# Autodesk Inventor assembly: Pelvis
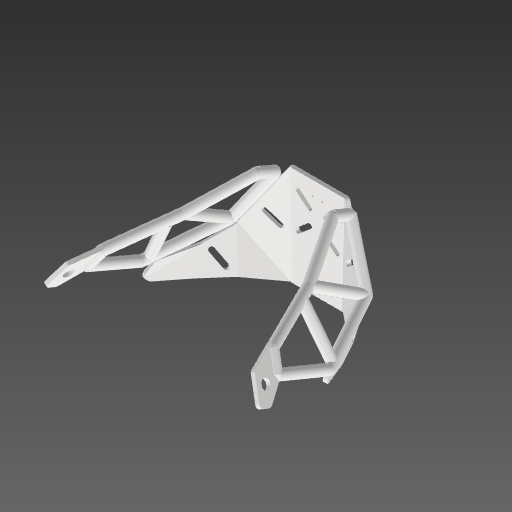
[picture p0: Inventor's stored thumbnail of the model, 512x512]
Saved by Autodesk Inventor 2020 (Build 240168000, 168)
## iProperties
Created: 2020-05-05
Part Number: Pelvis
Document SubType Name: Assembly
Designer: valer
Author: valer
## Documents named in this file (3)
- C:\Users\valer\Desktop\drummingrobot\src\Pelvis.iam
- C:\Users\valer\Desktop\drummingrobot\src\SpineLinkRoot.ipt
- C:\Users\valer\Desktop\drummingrobot\src\PelvisWing.ipt
## Components (3 placed, 2 different names)
1. SpineLinkRoot:1 — Mate:1, Mate:2
2. PelvisWing:1
3. PelvisWing:2
## Relationships (2: Mate 2)
- Mate:1: SpineLinkRoot:1
- Mate:2: SpineLinkRoot:1
